# Autodesk Inventor assembly: clock
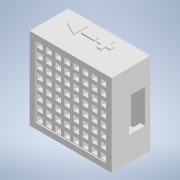
[picture p0: Inventor's stored thumbnail of the model, 180x180]
Saved by Autodesk Inventor 2020.1 (Build 241239000, 239)
## iProperties
Created: 2019-09-03
Part Number: clock
Document SubType Name: Assembly
Designer: matteo.spadetto-1
Author: matteo.spadetto-1
## Documents named in this file (9)
- C:\Users\matteo.spadetto-1\Desktop\Clock\clock.iam
- C:\Users\matteo.spadetto-1\Desktop\Clock\StandMatrix.ipt
- C:\Users\matteo.spadetto-1\Desktop\Clock\LedMatrix.ipt
- C:\Users\matteo.spadetto-1\Desktop\Clock\Case.ipt
- C:\Users\matteo.spadetto-1\Desktop\Clock\CaseBottom.ipt
- C:\Users\matteo.spadetto-1\Desktop\Clock\MinusBtn.ipt
- C:\Users\matteo.spadetto-1\Desktop\Clock\OkBtn.ipt
- C:\Users\matteo.spadetto-1\Desktop\Clock\PlusBtn.ipt
- C:\Users\matteo.spadetto-1\Desktop\Clock\StandBtn.ipt
## Components (8 placed, 8 different names)
1. StandMatrix:1 — Mate:1, Flush:1, Flush:2, Mate:2, Mate:3, Mate:4
2. LedMatrix:1 — Mate:1, Flush:1, Flush:2
3. Case:1 — Mate:2, Mate:3, Mate:4, Flush:3, Flush:4, Mate:5, Mate:8, Mate:11, Mate:14, Mate:15, Mate:16, Mate:17, Mate:18, Mate:19, Mate:20
4. CaseBottom:1 — Flush:3, Flush:4, Mate:5, Mate:22, Mate:23
5. MinusBtn:1 — Mate:11, Mate:15, Mate:16, Mate:21
6. OkBtn:1 — Mate:14, Mate:17, Mate:18
7. PlusBtn:1 — Mate:8, Mate:19, Mate:20
8. StandBtn:1 — Mate:21, Mate:22, Mate:23
## Relationships (21: Mate 17, Flush 4)
- Mate:1: StandMatrix:1 ↔ LedMatrix:1
- Flush:1: StandMatrix:1 ↔ LedMatrix:1
- Flush:2: StandMatrix:1 ↔ LedMatrix:1
- Mate:2: StandMatrix:1 ↔ Case:1
- Mate:3: StandMatrix:1 ↔ Case:1
- Mate:4: StandMatrix:1 ↔ Case:1
- Flush:3: Case:1 ↔ CaseBottom:1
- Flush:4: Case:1 ↔ CaseBottom:1
- Mate:5: Case:1 ↔ CaseBottom:1
- Mate:8: Case:1 ↔ PlusBtn:1
- Mate:11: Case:1 ↔ MinusBtn:1
- Mate:14: Case:1 ↔ OkBtn:1
- Mate:15 (0.1 mm): Case:1 ↔ MinusBtn:1
- Mate:16 (0.1 mm): Case:1 ↔ MinusBtn:1
- Mate:17 (0.1 mm): Case:1 ↔ OkBtn:1
- Mate:18 (0.1 mm): Case:1 ↔ OkBtn:1
- Mate:19 (0.1 mm): Case:1 ↔ PlusBtn:1
- Mate:20 (0.1 mm): Case:1 ↔ PlusBtn:1
- Mate:21 (5 mm): MinusBtn:1 ↔ StandBtn:1
- Mate:22: CaseBottom:1 ↔ StandBtn:1
- Mate:23 (1 mm): CaseBottom:1 ↔ StandBtn:1
